# Autodesk Inventor assembly: HF30
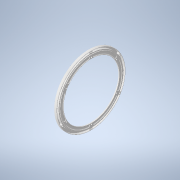
[picture p0: Inventor's stored thumbnail of the model, 180x180]
Saved by Autodesk Inventor 2022.3 (Build 263350000, 350)
## iProperties
Created: 2016-09-12
Part Number: HF30
Description: STEP AP203
Document SubType Name: Assembly
Designer: satot
Sending System: SolidWorks 2015
Preprocessor: SwSTEP 2.0
Title: SC210-11542_HF30_^[e[u_1.step
Revision Number: ANY
## Documents named in this file (3)
- C:\Users\YusukeKunita\Documents\GrabCAD\NHK2022\BasicParts\TurnTable\HF30\HF30.iam
- C:\Users\YusukeKunita\Documents\GrabCAD\NHK2022\BasicParts\TurnTable\HF30\SC210-11539_HF30_x[Xv[g.ipt
- C:\Users\YusukeKunita\Documents\GrabCAD\NHK2022\BasicParts\TurnTable\HF30\SC210-11540_HF30_gbvv[g.ipt
## Components (2 placed, 2 different names)
1. SC210-11539_HF30_x[Xv[g_1 — 回転:1
2. SC210-11540_HF30_gbvv[g_2 — 回転:1
## Relationships (1: RevoluteJoint 1)
- 回転:1 [RevoluteJoint] (14 mm): SC210-11539_HF30_x[Xv[g_1 ↔ SC210-11540_HF30_gbvv[g_2
